# Autodesk Inventor assembly: GP1-100
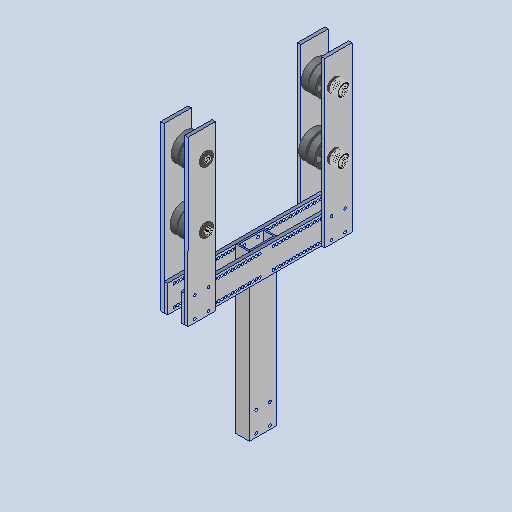
[picture p0: Inventor's stored thumbnail of the model, 512x512]
Saved by Autodesk Inventor 2023.4 (Build 274418000, 418)
## iProperties
Created: 2025-01-05
Part Number: GP1-100
Document SubType Name: Assembly
Designer: mavericks
Author: mavericks
## Documents named in this file (9)
- C:\Users\mavericks\Desktop\2025-ReefScape---CAD\Gripper\GP1-100.iam
- C:\Users\mavericks\Desktop\2025-ReefScape---CAD\Gripper\Gp1-001.ipt
- C:\Users\mavericks\Desktop\2025-ReefScape---CAD\Gripper\GP1-002.ipt
- C:\Users\mavericks\Desktop\2025-ReefScape---CAD\Gripper\GP1-003.ipt
- C:\Users\mavericks\Desktop\2025-ReefScape---CAD\COMMON PARTS\BEARINGS\10_25mm_3_8_ThunderHex_ID_x_0_875_OD_x_0_280_WD_Flanged_Bearing_217-5829.ipt
- C:\Users\mavericks\Desktop\2025-ReefScape---CAD\Gripper\GP1-004.ipt
- C:\Users\mavericks\Desktop\2025-ReefScape---CAD\Gripper\GP1-005.ipt
- C:\Users\mavericks\Desktop\2025-ReefScape---CAD\COMMON PARTS\PULLEYS\gt2\24T_GT2_375_HexBore_9mm_wide_Flanged_Pulley.ipt
- C:\Users\mavericks\Desktop\2025-ReefScape---CAD\COMMON PARTS\WHEELS\2_OD_Straight_Flex_Wheel_217-6354.ipt
## Components (31 placed, 8 different names)
1. GP1-002:1 — Insert:5, Insert:6, Insert:25, Insert:26
2. GP1-002:2 — Insert:19, Insert:21, Insert:27, Insert:28
3. GP1-002:3 — Insert:1, Insert:2, Insert:23, Insert:24
4. GP1-002:4 — Insert:20, Insert:22, Insert:29, Insert:30
5. Gp1-001:2 — Insert:1, Insert:2, Flush:1, Flush:2, Insert:9, Insert:12, Insert:15, Insert:29, Insert:30
6. Gp1-001:3 — Insert:5, Insert:6, Flush:1, Flush:2, Insert:10, Insert:11, Insert:13, Insert:14, Insert:16, Insert:17, Insert:18, Insert:27, Insert:28
7. GP1-003:1 — Insert:9, Insert:10, Insert:11, Insert:12, Insert:13, Insert:14, Insert:15, Insert:16, Insert:17, Insert:18
8. 10_25mm_3_8_ThunderHex_ID_x_0_875_OD_x_0_280_WD_Flanged_Bearing_217-5829:1 — Insert:19, Mate:8
9. 10_25mm_3_8_ThunderHex_ID_x_0_875_OD_x_0_280_WD_Flanged_Bearing_217-5829:2 — Insert:21, Mate:4, Mate:9
10. 10_25mm_3_8_ThunderHex_ID_x_0_875_OD_x_0_280_WD_Flanged_Bearing_217-5829:3 — Insert:20, Mate:1
11. 10_25mm_3_8_ThunderHex_ID_x_0_875_OD_x_0_280_WD_Flanged_Bearing_217-5829:4 — Insert:22
12. 10_25mm_3_8_ThunderHex_ID_x_0_875_OD_x_0_280_WD_Flanged_Bearing_217-5829:5 — Insert:26
13. 10_25mm_3_8_ThunderHex_ID_x_0_875_OD_x_0_280_WD_Flanged_Bearing_217-5829:6 — Insert:25
14. 10_25mm_3_8_ThunderHex_ID_x_0_875_OD_x_0_280_WD_Flanged_Bearing_217-5829:7 — Insert:24, Mate:5, Mate:13
15. 10_25mm_3_8_ThunderHex_ID_x_0_875_OD_x_0_280_WD_Flanged_Bearing_217-5829:8 — Insert:23, Mate:2, Mate:11
16. GP1-004:2 — Mate:1, Mate:7, Flush:3, Mate:22
17. GP1-004:3 — Mate:2, Mate:10, Flush:6, Mate:14, Mate:25
18. GP1-005:1 — Mate:4, Mate:6, Flush:4, Mate:17, Mate:23
19. GP1-005:2 — Mate:5, Mate:12, Flush:5, Mate:15, Mate:24
20. 24T_GT2_375_HexBore_9mm_wide_Flanged_Pulley:1 — Mate:10, Mate:11, Flush:6
21. 24T_GT2_375_HexBore_9mm_wide_Flanged_Pulley:2 — Mate:7, Mate:8, Flush:3, Mate:21
22. 24T_GT2_375_HexBore_9mm_wide_Flanged_Pulley:3 — Mate:12, Mate:13, Flush:5
23. 24T_GT2_375_HexBore_9mm_wide_Flanged_Pulley:4 — Mate:6, Mate:9, Flush:4
24. 2_OD_Straight_Flex_Wheel_217-6354:1 — Mate:17
25. 2_OD_Straight_Flex_Wheel_217-6354:2 — Mate:15
26. 2_OD_Straight_Flex_Wheel_217-6354:3 — Mate:14
27. 2_OD_Straight_Flex_Wheel_217-6354:4 — Mate:22
28. 2_OD_Straight_Flex_Wheel_217-6354:5 — Mate:21
29. 2_OD_Straight_Flex_Wheel_217-6354:6 — Mate:23
30. 2_OD_Straight_Flex_Wheel_217-6354:7 — Mate:25
31. 2_OD_Straight_Flex_Wheel_217-6354:8 — Mate:24
## Relationships (52: Insert 26, Mate 20, Flush 6)
- Insert:1: GP1-002:3 ↔ Gp1-001:2
- Insert:2: GP1-002:3 ↔ Gp1-001:2
- Insert:5: GP1-002:1 ↔ Gp1-001:3
- Insert:6: GP1-002:1 ↔ Gp1-001:3
- Flush:1: Gp1-001:2 ↔ Gp1-001:3
- Flush:2: Gp1-001:2 ↔ Gp1-001:3
- Insert:9: Gp1-001:2 ↔ GP1-003:1
- Insert:10: Gp1-001:3 ↔ GP1-003:1
- Insert:11: Gp1-001:3 ↔ GP1-003:1
- Insert:12: Gp1-001:2 ↔ GP1-003:1
- Insert:13: Gp1-001:3 ↔ GP1-003:1
- Insert:14: Gp1-001:3 ↔ GP1-003:1
- Insert:15: Gp1-001:2 ↔ GP1-003:1
- Insert:16: Gp1-001:3 ↔ GP1-003:1
- Insert:17: Gp1-001:3 ↔ GP1-003:1
- Insert:18: Gp1-001:3 ↔ GP1-003:1
- Insert:19: GP1-002:2 ↔ 10_25mm_3_8_ThunderHex_ID_x_0_875_OD_x_0_280_WD_Flanged_Bearing_217-5829:1
- Insert:20: GP1-002:4 ↔ 10_25mm_3_8_ThunderHex_ID_x_0_875_OD_x_0_280_WD_Flanged_Bearing_217-5829:3
- Insert:21: GP1-002:2 ↔ 10_25mm_3_8_ThunderHex_ID_x_0_875_OD_x_0_280_WD_Flanged_Bearing_217-5829:2
- Insert:22: GP1-002:4 ↔ 10_25mm_3_8_ThunderHex_ID_x_0_875_OD_x_0_280_WD_Flanged_Bearing_217-5829:4
- Insert:23: GP1-002:3 ↔ 10_25mm_3_8_ThunderHex_ID_x_0_875_OD_x_0_280_WD_Flanged_Bearing_217-5829:8
- Insert:24: GP1-002:3 ↔ 10_25mm_3_8_ThunderHex_ID_x_0_875_OD_x_0_280_WD_Flanged_Bearing_217-5829:7
- Insert:25: GP1-002:1 ↔ 10_25mm_3_8_ThunderHex_ID_x_0_875_OD_x_0_280_WD_Flanged_Bearing_217-5829:6
- Insert:26: GP1-002:1 ↔ 10_25mm_3_8_ThunderHex_ID_x_0_875_OD_x_0_280_WD_Flanged_Bearing_217-5829:5
- Mate:1: 10_25mm_3_8_ThunderHex_ID_x_0_875_OD_x_0_280_WD_Flanged_Bearing_217-5829:3 ↔ GP1-004:2
- Mate:2: 10_25mm_3_8_ThunderHex_ID_x_0_875_OD_x_0_280_WD_Flanged_Bearing_217-5829:8 ↔ GP1-004:3
- Mate:4: 10_25mm_3_8_ThunderHex_ID_x_0_875_OD_x_0_280_WD_Flanged_Bearing_217-5829:2 ↔ GP1-005:1
- Mate:5: 10_25mm_3_8_ThunderHex_ID_x_0_875_OD_x_0_280_WD_Flanged_Bearing_217-5829:7 ↔ GP1-005:2
- Mate:6: GP1-005:1 ↔ 24T_GT2_375_HexBore_9mm_wide_Flanged_Pulley:4
- Mate:7: GP1-004:2 ↔ 24T_GT2_375_HexBore_9mm_wide_Flanged_Pulley:2
- Mate:8: 10_25mm_3_8_ThunderHex_ID_x_0_875_OD_x_0_280_WD_Flanged_Bearing_217-5829:1 ↔ 24T_GT2_375_HexBore_9mm_wide_Flanged_Pulley:2
- Mate:9: 10_25mm_3_8_ThunderHex_ID_x_0_875_OD_x_0_280_WD_Flanged_Bearing_217-5829:2 ↔ 24T_GT2_375_HexBore_9mm_wide_Flanged_Pulley:4
- Flush:3: GP1-004:2 ↔ 24T_GT2_375_HexBore_9mm_wide_Flanged_Pulley:2
- Flush:4: GP1-005:1 ↔ 24T_GT2_375_HexBore_9mm_wide_Flanged_Pulley:4
- Mate:10: GP1-004:3 ↔ 24T_GT2_375_HexBore_9mm_wide_Flanged_Pulley:1
- Mate:11: 10_25mm_3_8_ThunderHex_ID_x_0_875_OD_x_0_280_WD_Flanged_Bearing_217-5829:8 ↔ 24T_GT2_375_HexBore_9mm_wide_Flanged_Pulley:1
- Mate:12: GP1-005:2 ↔ 24T_GT2_375_HexBore_9mm_wide_Flanged_Pulley:3
- Mate:13: 10_25mm_3_8_ThunderHex_ID_x_0_875_OD_x_0_280_WD_Flanged_Bearing_217-5829:7 ↔ 24T_GT2_375_HexBore_9mm_wide_Flanged_Pulley:3
- Flush:5: GP1-005:2 ↔ 24T_GT2_375_HexBore_9mm_wide_Flanged_Pulley:3
- Flush:6: GP1-004:3 ↔ 24T_GT2_375_HexBore_9mm_wide_Flanged_Pulley:1
- Mate:14: GP1-004:3 ↔ 2_OD_Straight_Flex_Wheel_217-6354:3
- Mate:15: GP1-005:2 ↔ 2_OD_Straight_Flex_Wheel_217-6354:2
- Mate:17: GP1-005:1 ↔ 2_OD_Straight_Flex_Wheel_217-6354:1
- Mate:21: 24T_GT2_375_HexBore_9mm_wide_Flanged_Pulley:2 ↔ 2_OD_Straight_Flex_Wheel_217-6354:5
- Mate:22: GP1-004:2 ↔ 2_OD_Straight_Flex_Wheel_217-6354:4
- Mate:23: GP1-005:1 ↔ 2_OD_Straight_Flex_Wheel_217-6354:6
- Mate:24: GP1-005:2 ↔ 2_OD_Straight_Flex_Wheel_217-6354:8
- Mate:25: GP1-004:3 ↔ 2_OD_Straight_Flex_Wheel_217-6354:7
- Insert:27: GP1-002:2 ↔ Gp1-001:3
- Insert:28: GP1-002:2 ↔ Gp1-001:3
- Insert:29: GP1-002:4 ↔ Gp1-001:2
- Insert:30: GP1-002:4 ↔ Gp1-001:2
